# Autodesk Inventor assembly: FAN_assembley
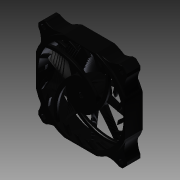
[picture p0: Inventor's stored thumbnail of the model, 180x180]
Saved by Autodesk Inventor 2015 (Build 190159000, 159)
## iProperties
Created: 2014-08-28
Part Number: FAN_assembley
Document SubType Name: Assembly
Designer: user
Author: user
## Documents named in this file (3)
- D:\WORK\PROTO\3D\P3301\FAN\FAN_assembley.iam
- D:\WORK\PROTO\3D\P3301\FAN\FAN_base.ipt
- D:\WORK\PROTO\3D\P3301\FAN\FAN.ipt
## Components (2 placed, 2 different names)
1. FAN_base:1 — Совмещение:1, Совмещение:3
2. FAN:1 — Совмещение:2, Совмещение:3
## Relationships (3: Mate 3)
- Совмещение:1 [Mate]: FAN_base:1
- Совмещение:2 [Mate]: FAN:1
- Совмещение:3 [Mate]: FAN_base:1 ↔ FAN:1
